# Autodesk Inventor assembly: lanceur
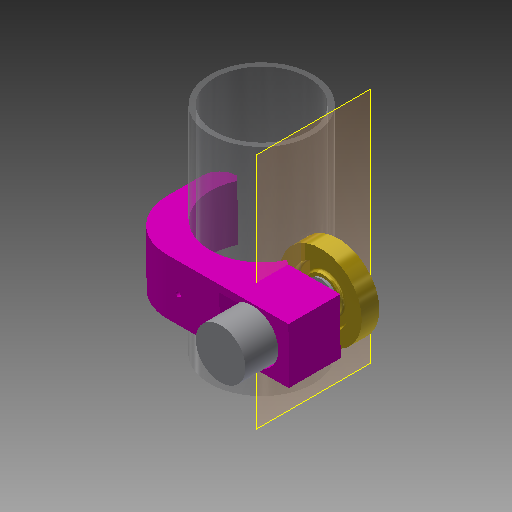
[picture p0: Inventor's stored thumbnail of the model, 512x512]
Saved by Autodesk Inventor 2017 (Build 210142000, 142)
## iProperties
Created: 2018-03-31
Part Number: lanceur
Document SubType Name: Assembly
Designer: franc
Author: franc
## Documents named in this file (7)
- C:\Users\franc\Desktop\EsialRobotik\Mecanique\2018\robot\traitement-eau\lanceur.iam
- C:\Users\franc\Desktop\EsialRobotik\Mecanique\2018\robot\traitement-eau\cylindre-lanceur.ipt
- C:\Users\franc\Desktop\EsialRobotik\Mecanique\2018\robot\traitement-eau\moteur.ipt
- C:\Users\franc\Desktop\EsialRobotik\Mecanique\composants\Roues\Banebot\T40_hub_40mm_1screw.ipt
- C:\Users\franc\Desktop\EsialRobotik\Mecanique\composants\Roues\Banebot\T40_Wheel_1_875in_x_0_5in.ipt
- C:\Users\franc\Desktop\EsialRobotik\Mecanique\2018\robot\traitement-eau\moyeu.ipt
- C:\Users\franc\Desktop\EsialRobotik\Mecanique\2018\robot\traitement-eau\support-moteur.ipt
## Components (6 placed, 6 different names)
1. cylindre-lanceur:1 — Placage:6, Tangente:1
2. moteur:1 — Placage:4, Placage:5, Affleurement:1, Placage:7, Placage:8, Tangente:1
3. T40_hub_40mm_1screw:1 — Placage:1, Placage:2, Placage:3, Placage:4, Affleurement:2
4. T40_Wheel_1_875in_x_0_5in:1 — Placage:1, Placage:2, Placage:3, Placage:6
5. moyeu:1 — Placage:5, Affleurement:1, Affleurement:2
6. support-moteur:1 — Placage:7, Placage:8
## Relationships (11: Mate 8, Flush 2, Tangent 1)
- Placage:1 [Mate]: T40_hub_40mm_1screw:1 ↔ T40_Wheel_1_875in_x_0_5in:1
- Placage:2 [Mate]: T40_hub_40mm_1screw:1 ↔ T40_Wheel_1_875in_x_0_5in:1
- Placage:3 [Mate]: T40_hub_40mm_1screw:1 ↔ T40_Wheel_1_875in_x_0_5in:1
- Placage:4 [Mate]: moteur:1 ↔ T40_hub_40mm_1screw:1
- Placage:5 [Mate]: moteur:1 ↔ moyeu:1
- Affleurement:1 [Flush]: moteur:1 ↔ moyeu:1
- Affleurement:2 [Flush]: T40_hub_40mm_1screw:1 ↔ moyeu:1
- Placage:6 [Mate] (1.5 mm): cylindre-lanceur:1 ↔ T40_Wheel_1_875in_x_0_5in:1
- Placage:7 [Mate]: moteur:1 ↔ support-moteur:1
- Placage:8 [Mate]: moteur:1 ↔ support-moteur:1
- Tangente:1 (-5 mm): cylindre-lanceur:1 ↔ moteur:1
